(part 1 of 3)
# Autodesk Inventor assembly: Ensamblaje2
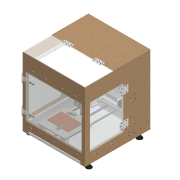
[picture p0: Inventor's stored thumbnail of the model, 180x180]
Saved by Autodesk Inventor 2020 (Build 240168000, 168)
## iProperties
Created: 2020-05-25
Part Number: Ensamblaje2
Document SubType Name: Assembly
Designer: Pipi
Author: Pipi
## Documents named in this file (110)
- C:\Users\Usuario\Desktop\Ensamble Ajuste Fino\Ensamblaje2.iam
- C:\Users\Usuario\Desktop\Ensamble Ajuste Fino\Culata.ipt
- C:\Users\Usuario\Desktop\Ensamble Ajuste Fino\Frente.ipt
- C:\Users\Usuario\Desktop\Ensamble Ajuste Fino\Lateral.ipt
- C:\Users\Usuario\Desktop\Ensamble Ajuste Fino\Soporte para Patas Regulables.ipt
- C:\Users\Usuario\Desktop\Ensamble Ajuste Fino\Pata regulable M6.ipt
- C:\Users\Usuario\Desktop\Ensamble Ajuste Fino\Guias de mesa.ipt
- C:\Users\Usuario\Desktop\Ensamble Ajuste Fino\Tornillo de mesa.ipt
- C:\Users\Usuario\Desktop\Ensamble Ajuste Fino\Buje para Tornillo.ipt
- C:\Users\Usuario\Desktop\Ensamble Ajuste Fino\Mesa.ipt
- C:\Users\Usuario\Desktop\Ensamble Ajuste Fino\Soporte de Buje.ipt
- C:\Users\Usuario\Desktop\Ensamble Ajuste Fino\Soporte de tuerca de mesa.ipt
- C:\Users\Usuario\Desktop\Ensamble Ajuste Fino\Buje para Guía.ipt
- C:\Users\Usuario\Desktop\Ensamble Ajuste Fino\Columna Derecha.ipt
- C:\Users\Usuario\Desktop\Ensamble Ajuste Fino\Columna Izquierda.ipt
- C:\Users\Usuario\Desktop\Ensamble Ajuste Fino\Guías de Vínculo Cabezal.ipt
- C:\Users\Usuario\Desktop\Ensamble Ajuste Fino\Tornillo de Vínculo Cabezal.ipt
- C:\Users\Usuario\Desktop\Ensamble Ajuste Fino\Travesaño Estructural.ipt
- C:\Users\Usuario\Desktop\Ensamble Ajuste Fino\Vertical Vìnculo Cabezal.ipt
- C:\Users\Usuario\Desktop\Ensamble Ajuste Fino\Bloque - Vinculo Cabezal.ipt
- C:\Users\Usuario\Desktop\Ensamble Ajuste Fino\Techo, Vínculo Cabezal.ipt
- C:\Users\Usuario\Desktop\Ensamble Ajuste Fino\Piso, Vínculo Cabezal.ipt
- C:\Users\Usuario\Desktop\Ensamble Ajuste Fino\Separador de Bujes.ipt
- C:\Users\Usuario\Desktop\Ensamble Ajuste Fino\Tapa para Buje.ipt
- C:\Users\Usuario\Desktop\Ensamble Ajuste Fino\motor DC.ipt
- C:\Users\Usuario\Desktop\Ensamble Ajuste Fino\Soporte de Motor.ipt
- C:\Users\Usuario\Desktop\Ensamble Ajuste Fino\Acople de soporte de motor.ipt
- C:\Users\Usuario\Desktop\Ensamble Ajuste Fino\Guías de Soporte de Motor.ipt
- C:\Users\Usuario\Desktop\Ensamble Ajuste Fino\Tornillo de Soporte de Motor.ipt
- C:\Users\Usuario\Desktop\Ensamble Ajuste Fino\Buje de Soporte de Motor.ipt
- C:\Users\Usuario\Desktop\Ensamble Ajuste Fino\Tornillo allen cabeza cilindrica M6x20mm.ipt
- C:\Users\Usuario\Desktop\Ensamble Ajuste Fino\Arandela Grower m6.ipt
- C:\Users\Usuario\Desktop\Ensamble Ajuste Fino\Tornillo Allen cabeza cilindrica M4x30mm.ipt
- C:\Users\Usuario\Desktop\Ensamble Ajuste Fino\Tornillo Allen cabeza cilindrica M4x16mm.ipt
- C:\Users\Usuario\Desktop\Ensamble Ajuste Fino\Nema 17.iam
- C:\Users\Usuario\Desktop\Ensamble Ajuste Fino\Acople de Motor PAP.ipt
- C:\Users\Usuario\Desktop\Ensamble Ajuste Fino\Tornillo Allen cabeza fresada M4x16mm.ipt
- C:\Users\Usuario\Desktop\Ensamble Ajuste Fino\Espaciador Sub Inferior.ipt
- C:\Users\Usuario\Desktop\Ensamble Ajuste Fino\Techo Espaciador Sub. Inferior.ipt
- C:\Users\Usuario\Desktop\Ensamble Ajuste Fino\Tornillo Allen cabeza botón M6x20mm.ipt
- C:\Users\Usuario\Desktop\Ensamble Ajuste Fino\Tornillo Allen cabeeza botón M3x8mm.ipt
- C:\Users\Usuario\Desktop\Ensamble Ajuste Fino\Espaciador Derecho.ipt
- C:\Users\Usuario\Desktop\Ensamble Ajuste Fino\Espaciador Izquierdo.ipt
- C:\Users\Usuario\Desktop\Ensamble Ajuste Fino\Techo Espaciador.ipt
- C:\Users\Usuario\Desktop\Ensamble Ajuste Fino\Tornillo Allen cabeza cilindrica M4x45mm.ipt
- C:\Users\Usuario\Desktop\Ensamble Ajuste Fino\Tornillo Allen cabeza cilindrica M4x20mm.ipt
- C:\Users\Usuario\Desktop\Ensamble Ajuste Fino\Tornillo Allen cabeza botón M4x20mm.ipt
- C:\Users\Usuario\Desktop\Ensamble Ajuste Fino\Final de Carrera.ipt
- C:\Users\Usuario\Desktop\Ensamble Ajuste Fino\Soporte de Final de Carrera - Eje X.ipt
- C:\Users\Usuario\Desktop\Ensamble Ajuste Fino\Tornillo Gusano Allen M3x16mm.ipt
- C:\Users\Usuario\Desktop\Ensamble Ajuste Fino\Herramienta Punta de Lanza.ipt
- C:\Users\Usuario\Desktop\Ensamble Ajuste Fino\Tornillo Allen cabeza botón M4x10mm.ipt
- C:\Users\Usuario\Desktop\Ensamble Ajuste Fino\Tuerca de mesa.ipt
- C:\Users\Usuario\Desktop\Ensamble Ajuste Fino\Arandela Plana Tipo A DIN 125 - M4.ipt
- C:\Users\Usuario\Desktop\Ensamble Ajuste Fino\Chaponete.ipt
- C:\Users\Usuario\Desktop\Ensamble Ajuste Fino\placa pcb 100x150mm.ipt
- C:\Users\Usuario\Desktop\Ensamble Ajuste Fino\Tornillo Allen cabeza fresada M3x20mm.ipt
- C:\Users\Usuario\Desktop\Ensamble Ajuste Fino\Arandela plana tipo A DIN 125 M6.ipt
- C:\Users\Usuario\Desktop\Ensamble Ajuste Fino\Tornillo Allen cabeza botón M6x16mm.ipt
- C:\Users\Usuario\Desktop\Ensamble Ajuste Fino\Tornillo allen cabeza boton M8x16mm.ipt
- C:\Users\Usuario\Desktop\Ensamble Ajuste Fino\Arandela Grower M8.ipt
- C:\Users\Usuario\Desktop\Ensamble Ajuste Fino\Soporte de Final de Carrera - Eje Y.ipt
- C:\Users\Usuario\Desktop\Ensamble Ajuste Fino\Placa de Mecanizado.ipt
- C:\Users\Usuario\Desktop\Ensamble Ajuste Fino\Esquina de bandeja.ipt
- C:\Users\Usuario\Desktop\Ensamble Ajuste Fino\Tornillo Allen cabeza cilindrica M4x35mm.ipt
- C:\Users\Usuario\Desktop\Ensamble Ajuste Fino\Tornillo Allen cabeza cilindrica M2x16mm.ipt
- C:\Users\Usuario\Desktop\Ensamble Ajuste Fino\Tapa de Mandril.ipt
- C:\Users\Usuario\Desktop\Ensamble Ajuste Fino\Remache POP Abierto con Rotura de Vástago D4.ipt
- C:\Users\Usuario\Desktop\Ensamble Ajuste Fino\Tornillo Allen gusano M6 para Motor.ipt
- C:\Users\Usuario\Desktop\Ensamble Ajuste Fino\Guía de Bandeja Der..ipt
- C:\Users\Usuario\Desktop\Ensamble Ajuste Fino\Guía de Bandeja Izq..ipt
- C:\Users\Usuario\Desktop\Ensamble Ajuste Fino\Bandeja.ipt
- C:\Users\Usuario\Desktop\Ensamble Ajuste Fino\Opción B - Sujeción Motor Paso a Paso\NEMA 17 90°.ipt
- C:\Users\Usuario\Desktop\Ensamble Ajuste Fino\Opción B - Sujeción Motor Paso a Paso\Estante para Soporte de Motor PaP.ipt
- C:\Users\Usuario\Desktop\Ensamble Ajuste Fino\Frente Carcasa.ipt
- C:\Users\Usuario\Desktop\Ensamble Ajuste Fino\Lateral Derecho Carcasa.ipt
- C:\Users\Usuario\Desktop\Ensamble Ajuste Fino\Lateral Izquierdo Carcasa.ipt
- C:\Users\Usuario\Desktop\Ensamble Ajuste Fino\Techo Carcasa.ipt
- C:\Users\Usuario\Desktop\Ensamble Ajuste Fino\Culata Carcaza.ipt
- C:\Users\Usuario\Desktop\Ensamble Ajuste Fino\Chapon.ipt
- C:\Users\Usuario\Desktop\Ensamble Ajuste Fino\Separador Lateral.ipt
- C:\Users\Usuario\Desktop\Ensamble Ajuste Fino\Cielo raso.ipt
- C:\Users\Usuario\Desktop\Ensamble Ajuste Fino\Puerta Lateral Izquierda.ipt
- C:\Users\Usuario\Desktop\Ensamble Ajuste Fino\Ala 1 Bisagra tipo Libro Grande.ipt
- C:\Users\Usuario\Desktop\Ensamble Ajuste Fino\Ala 2 Bisagra tipo Libro Grande.ipt
- C:\Users\Usuario\Desktop\Ensamble Ajuste Fino\Ala 1 Bisagra tipo T.ipt
- C:\Users\Usuario\Desktop\Ensamble Ajuste Fino\Ala 2 Bisagra tipo T.ipt
- C:\Users\Usuario\Desktop\Ensamble Ajuste Fino\Distanciador para Laterales.ipt
- C:\Users\Usuario\Desktop\Ensamble Ajuste Fino\Ala 1 Bisagra tipo Libro Chica.ipt
- C:\Users\Usuario\Desktop\Ensamble Ajuste Fino\Ala 2 Bisagra tipo Libro Chica.ipt
- C:\Users\Usuario\Desktop\Ensamble Ajuste Fino\Soporte L.ipt
- C:\Users\Usuario\Desktop\Ensamble Ajuste Fino\Tuerca remache m4.ipt
- C:\Users\Usuario\Desktop\Ensamble Ajuste Fino\Chapa Base.ipt
- C:\Users\Usuario\Documents\Inventor\Content Center Files\R2020\en-US\ISO 4032(2)\ISO 4032 - M6 - ISO.ipt
- C:\Users\Usuario\Documents\Inventor\Content Center Files\R2020\en-US\ISO 4032(2)\ISO 4032 - M4 - ISO.ipt
- C:\Users\Usuario\Desktop\Ensamble Ajuste Fino\Tornillo allen cabeza boton M5x10mm.ipt
- C:\Users\Usuario\Desktop\Ensamble Ajuste Fino\Arandela plana tipo A DIN 125-M5.ipt
- C:\Users\Usuario\Documents\Inventor\Content Center Files\R2020\en-US\ISO 4032(2)\ISO 4032 - M5 - ISO.ipt
- C:\Users\Usuario\Desktop\Ensamble Ajuste Fino\Tornillo allen cabeza boton M5x16mm.ipt
- C:\Users\Usuario\Desktop\Ensamble Ajuste Fino\Puerta Frontal.ipt
- C:\Users\Usuario\Desktop\Ensamble Ajuste Fino\Puerta Lateral Derecha.ipt
- C:\Users\Usuario\Desktop\Ensamble Ajuste Fino\Puerta de Inspección.ipt
- C:\Users\Usuario\Desktop\Ensamble Ajuste Fino\Soporte para culata carcasa.ipt
- C:\Users\Usuario\Desktop\Ensamble Ajuste Fino\Tornillo Allen cabeza botón M4x16mm.ipt
- C:\Users\Usuario\Documents\Inventor\Content Center Files\R2020\en-US\ISO 4032(2)\ISO 4032 - M2 - ISO.ipt
- C:\Users\Usuario\Documents\Inventor\Content Center Files\R2020\en-US\ISO 4032(2)\ISO 4032 - M3 - ISO.ipt
- C:\Users\Usuario\Desktop\Ensamble Ajuste Fino\Kit de sujecion 2.ipt
- C:\Users\Usuario\Desktop\Ensamble Ajuste Fino\Kit sugecion 1.ipt
- C:\Users\Usuario\Desktop\Ensamble Ajuste Fino\Eslabon cadena portacable.ipt
- C:\Users\Usuario\Desktop\Ensamble Ajuste Fino\Tornillo Allen cabeeza botón M3x16mm.ipt
## Components (623 placed, 109 different names)
1. Culata:1 — Coincidencia:4, Coincidencia:91, Coincidencia:92, Coincidencia:93, Coincidencia:94, Coincidencia:95, Coincidencia:96, Coincidencia:148, Nivelación:20, Coincidencia:186, Coincidencia:220, Mate:275, Nivelación:38, Coincidencia:292, Insertar:469, Insertar:470
2. Frente:1 — Coincidencia:21, Coincidencia:22, Nivelación:12, Nivelación:16, Nivelación:17, Coincidencia:154, Insertar:236, Insertar:285, Coincidencia:193, Insertar:286, Coincidencia:274, Coincidencia:400
3. Lateral:1 — Coincidencia:4, Insertar:35, Insertar:36, Insertar:37, Insertar:38, Insertar:71, Insertar:72, Coincidencia:89, Coincidencia:90, Nivelación:12, Insertar:236, Nivelación:39, Mate:301, Mate:302, Mate:303, Coincidencia:385, Nivelación:58, Insertar:487, Insertar:488, Insertar:489
4. Lateral:2 — Nivelación:16, Nivelación:17, Coincidencia:154, Insertar:234, Insertar:235, Insertar:237, Insertar:238, Insertar:239, Coincidencia:155, Insertar:254, Coincidencia:170, Insertar:308, Mate:304, Mate:305, Mate:306, Coincidencia:383, Nivelación:57, Insertar:490, Insertar:491, Insertar:492
5. Soporte para Patas Regulables:1 — Insertar:2, Insertar:72, Coincidencia:90, Insertar:77, Insertar:78
6. Soporte para Patas Regulables:2 — Insertar:3, Insertar:73, Insertar:74, Insertar:239
7. Soporte para Patas Regulables:3 — Insertar:4, Insertar:75, Insertar:76, Insertar:254, Coincidencia:170
8. Soporte para Patas Regulables:4 — Insertar:1, Insertar:71, Coincidencia:89, Insertar:79, Insertar:80
9. Pata regulable M6:1 — Insertar:1
10. Pata regulable M6:2 — Insertar:2
11. Pata regulable M6:3 — Insertar:3
12. Pata regulable M6:4 — Insertar:4
13. Guias de mesa:1 — Insertar:285, Coincidencia:190, Coincidencia:212, Insertar:324, Insertar:330
14. Guias de mesa:2 — Coincidencia:193, Insertar:286, Coincidencia:194, Insertar:323, Insertar:329
15. Tornillo de mesa:1 — Insertar:278, Coincidencia:216
16. Buje para Tornillo:1 — Coincidencia:21, Coincidencia:22, Insertar:278
17. Mesa:1 — Coincidencia:197, Coincidencia:198, Coincidencia:200, Coincidencia:203, Coincidencia:205, Coincidencia:206, Coincidencia:208, Coincidencia:209, Coincidencia:210, Coincidencia:217, Coincidencia:218, Coincidencia:274, Mate:275, Nivelación:36, Coincidencia:280, Nivelación:37, Mate:363, Mate:364, Mate:368, Mate:369, Mate:370, Mate:371
18. Soporte de Buje:1 — Coincidencia:211, Nivelación:22, Coincidencia:218, Insertar:299, Insertar:300, Insertar:301, Insertar:302, Coincidencia:251, Coincidencia:256
19. Soporte de Buje:2 — Coincidencia:213, Nivelación:21, Coincidencia:217, Insertar:291, Insertar:292, Insertar:293, Insertar:294, Coincidencia:252, Coincidencia:254
20. Soporte de Buje:3 — Coincidencia:198, Coincidencia:203, Coincidencia:206, Coincidencia:215, Nivelación:24, Insertar:287, Insertar:288, Insertar:289, Insertar:290, Coincidencia:253, Coincidencia:255
21. Soporte de Buje:4 — Coincidencia:197, Coincidencia:200, Coincidencia:205, Coincidencia:214, Nivelación:23, Insertar:295, Insertar:296, Insertar:297, Insertar:298, Coincidencia:250, Coincidencia:257
22. Soporte de tuerca de mesa:1 — Coincidencia:208, Coincidencia:209, Coincidencia:210, Coincidencia:216, Insertar:303, Insertar:304, Insertar:305, Insertar:306, Insertar:307, Coincidencia:219, Coincidencia:423, Nivelación:60
23. Buje para Guía:1 — Coincidencia:212, Coincidencia:213, Nivelación:21, Insertar:341, Insertar:344
24. Buje para Guía:2 — Coincidencia:190, Coincidencia:211, Nivelación:22, Insertar:346, Insertar:349
25. Buje para Guía:3 — Coincidencia:215, Nivelación:24, Insertar:342, Insertar:343
26. Buje para Guía:4 — Coincidencia:194, Coincidencia:214, Nivelación:23, Insertar:340, Insertar:345
27. Columna Derecha:1 — Coincidencia:40, Coincidencia:41, Coincidencia:44, Nivelación:7, Coincidencia:46, Nivelación:8, Insertar:128, Insertar:129, Insertar:170, Insertar:172, Insertar:173, Coincidencia:116, Insertar:174, Insertar:175, Insertar:205, Insertar:206, Insertar:207, Insertar:208, Insertar:237, Insertar:238, Insert:442, Mate:348, Flush:42, Coincidencia:384
28. Columna Izquierda:1 — Coincidencia:37, Coincidencia:42, Coincidencia:43, Coincidencia:45, Coincidencia:47, Coincidencia:48, Insertar:126, Insertar:127, Coincidencia:126, Coincidencia:127, Coincidencia:128, Insertar:201, Insertar:202, Insertar:203, Insertar:204, Coincidencia:386
29. Guías de Vínculo Cabezal:1 — Coincidencia:46, Nivelación:8, Coincidencia:64, Coincidencia:65, Coincidencia:66, Coincidencia:73, Coincidencia:74, Insertar:334, Insertar:338
30. Guías de Vínculo Cabezal:2 — Coincidencia:45, Nivelación:7, Coincidencia:61, Coincidencia:62, Coincidencia:63, Coincidencia:71, Coincidencia:72, Insertar:332, Insertar:336
31. Tornillo de Vínculo Cabezal:1 — Insertar:17, Coincidencia:117, Insertar:176, Coincidencia:173
32. Travesaño Estructural:1 — Coincidencia:37, Coincidencia:40, Coincidencia:41, Coincidencia:42, Coincidencia:43, Coincidencia:44, Insertar:747, Insertar:748, Insertar:749, Insertar:750
33. Buje para Tornillo:2 — Coincidencia:47, Coincidencia:48, Insertar:17
34. Vertical Vìnculo Cabezal:1 — Coincidencia:53, Coincidencia:54, Coincidencia:55, Coincidencia:56, Insertar:138, Insertar:139, Insertar:140, Insertar:141, Insertar:142, Insertar:143, Insertar:144, Insertar:145, Coincidencia:118, Coincidencia:120
35. Bloque - Vinculo Cabezal:1 — Coincidencia:118, Coincidencia:119, Coincidencia:120, Insertar:177, Insertar:178, Insertar:179, Insertar:180, Insertar:181, Insertar:182, Coincidencia:125, Coincidencia:139, Coincidencia:171, Coincidencia:172, Insertar:255, Coincidencia:174, Insertar:852, Insertar:853
36. Techo, Vínculo Cabezal:1 — Coincidencia:55, Coincidencia:56, Coincidencia:105, Coincidencia:106, Coincidencia:107, Coincidencia:108, Coincidencia:109, Coincidencia:110, Coincidencia:119, Insertar:279, Insertar:280, Insertar:364, Insertar:365, Insertar:366, Insertar:367, Coincidencia:271, Insertar:411, Coincidencia:291
37. Piso, Vínculo Cabezal:1 — Coincidencia:53, Coincidencia:54, Coincidencia:79, Coincidencia:80, Insertar:368, Insertar:369, Insertar:370, Insertar:371, Coincidencia:272
38. Buje para Guía:5 — Coincidencia:64, Coincidencia:70, Insertar:178
39. Buje para Guía:6 — Coincidencia:66, Coincidencia:69
40. Buje para Guía:7 — Coincidencia:62, Coincidencia:68, Insertar:177
41. Buje para Guía:8 — Coincidencia:61, Coincidencia:67
42. Separador de Bujes:1 — Coincidencia:65, Coincidencia:69, Coincidencia:70
43. Separador de Bujes:2 — Coincidencia:63, Coincidencia:67, Coincidencia:68
44. Tapa para Buje:1 — Coincidencia:72, Insertar:148, Insertar:149, Insertar:181
45. Tapa para Buje:2 — Coincidencia:74, Insertar:154, Insertar:155, Insertar:180
46. Tapa para Buje:3 — Coincidencia:73, Insertar:150, Insertar:151, Insertar:182
47. Tapa para Buje:4 — Coincidencia:71, Insertar:152, Insertar:153, Insertar:179
48. motor DC:1 — Coincidencia:270, Nivelación:31, Coincidencia:273, Nivelación:32, Mate:294, Mate:295
49. Acople de soporte de motor:1 — Coincidencia:263, Coincidencia:264, Insertar:389, Coincidencia:265, Insertar:390, Coincidencia:266, Insertar:391, Coincidencia:267, Insertar:392, Coincidencia:268, Insertar:393, Insertar:394, Insertar:395, Insertar:396, Insertar:397
50. Guías de Soporte de Motor:1 — Coincidencia:180, Insertar:280, Insertar:381, Insertar:383, Coincidencia:259, Coincidencia:263
51. Guías de Soporte de Motor:2 — Coincidencia:182, Insertar:279, Insertar:380, Insertar:382, Coincidencia:258, Coincidencia:264
52. Buje para Tornillo:3 — Coincidencia:79, Coincidencia:80, Insertar:24
53. Tornillo de Soporte de Motor:1 — Insertar:24, Coincidencia:290, Insertar:410
54. Buje de Soporte de Motor:1 — Insertar:266, Coincidencia:258, Insertar:391, Coincidencia:272
55. Buje de Soporte de Motor:2 — Coincidencia:180, Insertar:268, Insertar:390
56. Tornillo allen cabeza cilindrica M6x20mm:5 — Insertar:235
57. Tornillo allen cabeza cilindrica M6x20mm:6
58. Tornillo allen cabeza cilindrica M6x20mm:7 — Insertar:308, Coincidencia:220
59. Tornillo allen cabeza cilindrica M6x20mm:10 — Insertar:38
60. Tornillo allen cabeza cilindrica M6x20mm:15 — Insertar:37, Coincidencia:148
61. Tornillo allen cabeza cilindrica M6x20mm:16 — Insertar:35
62. Tornillo allen cabeza cilindrica M6x20mm:17 — Insertar:36
63. Tornillo allen cabeza cilindrica M6x20mm:20 — Insertar:234
64. Arandela Grower m6:1 — Insertar:320, Insert:429
65. Arandela Grower m6:2 — Insertar:322, Insert:428
66. Arandela Grower m6:3 — Insertar:326, Insert:427
67. Arandela Grower m6:4 — Insertar:328, Insert:426
68. Tornillo Allen cabeza cilindrica M4x30mm:1 — Insertar:290
69. Tornillo Allen cabeza cilindrica M4x30mm:2 — Insertar:291
70. Tornillo Allen cabeza cilindrica M4x30mm:3 — Insertar:299
71. Tornillo Allen cabeza cilindrica M4x30mm:4 — Insertar:301
72. Tornillo Allen cabeza cilindrica M4x30mm:5 — Insertar:298
73. Tornillo Allen cabeza cilindrica M4x30mm:6 — Insertar:287
74. Tornillo Allen cabeza cilindrica M4x30mm:7 — Insertar:294
75. Tornillo Allen cabeza cilindrica M4x30mm:8 — Insertar:302
76. Tornillo Allen cabeza cilindrica M4x30mm:9 — Insertar:288
77. Tornillo Allen cabeza cilindrica M4x30mm:10 — Insertar:300
78. Tornillo Allen cabeza cilindrica M4x30mm:15 — Insertar:293
79. Tornillo Allen cabeza cilindrica M4x30mm:16 — Insertar:292
80. Tornillo Allen cabeza cilindrica M4x30mm:17 — Insertar:296
81. Tornillo Allen cabeza cilindrica M4x30mm:18 — Insertar:289
82. Tornillo Allen cabeza cilindrica M4x30mm:19 — Insertar:297
83. Tornillo Allen cabeza cilindrica M4x30mm:20 — Insertar:295
84. Tornillo Allen cabeza cilindrica M4x16mm:1 — Insertar:83, Coincidencia:99
85. Tornillo Allen cabeza cilindrica M4x16mm:2 — Insertar:86
86. Tornillo Allen cabeza cilindrica M4x16mm:3 — Insertar:84
87. Tornillo Allen cabeza cilindrica M4x16mm:4 — Insertar:306
88. Tornillo Allen cabeza cilindrica M4x16mm:5 — Insertar:303
89. Tornillo Allen cabeza cilindrica M4x16mm:6 — Insertar:85
90. Nema 17:1 [sub-assembly] — Insertar:82, Coincidencia:99
91. Nema 17:2 [sub-assembly] — Coincidencia:116, Insertar:174, Insertar:175, Coincidencia:117, Mate:345, Mate:346, Mate:347
92. Nema 17:3 [sub-assembly] — Coincidencia:115, Insertar:169, Coincidencia:290
93. Acople de Motor PAP:2 — Insertar:176, Coincidencia:125
94. Acople de Motor PAP:1 — Nivelación:20, Coincidencia:186
95. Acople de Motor PAP:3 — Coincidencia:115, Insertar:410
96. Tornillo Allen cabeza fresada M4x16mm:1 — Insertar:77
97. Tornillo Allen cabeza fresada M4x16mm:2 — Insertar:78
98. Tornillo Allen cabeza fresada M4x16mm:3 — Insertar:79
99. Tornillo Allen cabeza fresada M4x16mm:4 — Insertar:74, Coincidencia:155
100. Tornillo Allen cabeza fresada M4x16mm:5 — Insertar:80
101. Tornillo Allen cabeza fresada M4x16mm:6 — Insertar:76
102. Tornillo Allen cabeza fresada M4x16mm:7 — Insertar:75
103. Tornillo Allen cabeza fresada M4x16mm:8 — Insertar:73
104. Espaciador Sub Inferior:1 — Coincidencia:92, Coincidencia:93, Coincidencia:94, Coincidencia:97, Insertar:91
105. Espaciador Sub Inferior:2 — Coincidencia:91, Coincidencia:95, Coincidencia:96, Mate:293
106. Techo Espaciador Sub. Inferior:1 — Insertar:82, Insertar:83, Insertar:84, Insertar:85, Insertar:86, Coincidencia:97, Insertar:91, Insert:412, Insert:413, Insert:414, Insert:415
107. Tornillo Allen cabeza cilindrica M4x16mm:7 — Insertar:305
108. Tornillo Allen cabeza cilindrica M4x16mm:8 — Insertar:304
109. Arandela Grower m6:5 — Insertar:372, Insertar:373
110. Arandela Grower m6:6 — Insertar:374, Insertar:375
111. Arandela Grower m6:7 — Insertar:109, Insertar:331
112. Arandela Grower m6:8 — Insertar:124, Insertar:128
113. Arandela Grower m6:9 — Insertar:103, Insertar:337
114. Arandela Grower m6:10 — Insertar:107, Insertar:333
115. Arandela Grower m6:11 — Insertar:122, Insertar:127
116. Arandela Grower m6:12 — Insertar:125, Insertar:129
117. Arandela Grower m6:13 — Insertar:100, Insertar:335
118. Arandela Grower m6:14 — Insertar:123, Insertar:126
119. Arandela Grower m6:15 — Insertar:378, Insertar:379
120. Arandela Grower m6:16 — Insertar:376, Insertar:377
121. Tornillo Allen cabeza botón M6x20mm:3 — Insertar:100
122. Tornillo Allen cabeza botón M6x20mm:4 — Insertar:107
123. Tornillo Allen cabeza botón M6x20mm:5 — Insertar:374
124. Tornillo Allen cabeza botón M6x20mm:6 — Insertar:109
125. Tornillo Allen cabeza botón M6x20mm:7 — Insertar:372
126. Tornillo Allen cabeza botón M6x20mm:8 — Insertar:103
127. Tornillo Allen cabeza botón M6x20mm:9 — Insertar:376
128. Tornillo Allen cabeza botón M6x20mm:10 — Insertar:378
129. Tornillo Allen cabeza botón M6x20mm:11 — Insertar:122
130. Tornillo Allen cabeza botón M6x20mm:12 — Insertar:124
131. Tornillo Allen cabeza botón M6x20mm:18 — Insertar:138
132. Tornillo Allen cabeza botón M6x20mm:20 — Insertar:125
133. Tornillo Allen cabeza botón M6x20mm:21 — Insertar:123
134. Tornillo Allen cabeza botón M6x20mm:22 — Insertar:144
135. Tornillo Allen cabeza botón M6x20mm:23 — Insertar:143
136. Tornillo Allen cabeza botón M6x20mm:24 — Insertar:140
137. Tornillo Allen cabeza botón M6x20mm:25 — Insertar:139
138. Tornillo Allen cabeza botón M6x20mm:26 — Insertar:145
139. Tornillo Allen cabeza botón M6x20mm:27 — Insertar:142
140. Tornillo Allen cabeza botón M6x20mm:28 — Insertar:141
141. Tornillo Allen cabeeza botón M3x8mm:1 — Insertar:153
142. Tornillo Allen cabeeza botón M3x8mm:2 — Insertar:150
143. Tornillo Allen cabeeza botón M3x8mm:3 — Insertar:152
144. Tornillo Allen cabeeza botón M3x8mm:4 — Insertar:154
145. Tornillo Allen cabeeza botón M3x8mm:5 — Insertar:155
146. Tornillo Allen cabeeza botón M3x8mm:6 — Insertar:151
147. Tornillo Allen cabeeza botón M3x8mm:7 — Insertar:148
148. Tornillo Allen cabeeza botón M3x8mm:8 — Insertar:149
149. Espaciador Derecho:1 — Coincidencia:108, Coincidencia:109, Coincidencia:110, Coincidencia:112, Coincidencia:113
150. Espaciador Izquierdo:1 — Coincidencia:105, Coincidencia:106, Coincidencia:107, Coincidencia:111, Coincidencia:114
151. Techo Espaciador:1 — Coincidencia:111, Coincidencia:112, Coincidencia:113, Coincidencia:114, Insertar:165, Insertar:166, Insertar:167, Insertar:168, Insertar:169, Insertar:185, Insertar:186, Insertar:187, Insertar:217, Insertar:218, Insertar:219, Insertar:220
152. Tornillo Allen cabeza cilindrica M4x45mm:1 — Insertar:186
153. Tornillo Allen cabeza cilindrica M4x45mm:3 — Insertar:185
154. Tornillo Allen cabeza cilindrica M4x45mm:4 — Insertar:187
155. Tornillo Allen cabeza cilindrica M4x20mm:1 — Insertar:167
156. Tornillo Allen cabeza cilindrica M4x20mm:2 — Insertar:166
157. Tornillo Allen cabeza cilindrica M4x20mm:3 — Insertar:165
158. Tornillo Allen cabeza cilindrica M4x20mm:4 — Insertar:168
159. Tornillo Allen cabeza botón M4x20mm:3 — Insertar:173
160. Tornillo Allen cabeza botón M4x20mm:4 — Insertar:172
161. Tornillo Allen cabeza botón M4x20mm:5 — Insertar:170
162. Final de Carrera:1 — Insertar:398, Coincidencia:277, Insert:420, Insert:421
163. Final de Carrera:2 — Coincidencia:129, Coincidencia:130, Coincidencia:131, Coincidencia:139, Insert:418, Insert:419
164. Final de Carrera:3 — Insertar:411, Coincidencia:291, Insert:416, Insert:417
165. Soporte de Final de Carrera - Eje X:1 — Coincidencia:126, Coincidencia:127, Coincidencia:128, Coincidencia:129, Coincidencia:130, Coincidencia:131, Insertar:213, Insertar:214, Coincidencia:420, Coincidencia:422
166. Arandela Grower m6:17 — Insertar:206, Insert:432
167. Arandela Grower m6:18 — Insertar:208, Insert:433
168. Arandela Grower m6:19 — Insertar:203, Insert:424
169. Arandela Grower m6:20 — Insertar:202, Insert:425
170. Arandela Grower m6:21 — Insertar:201, Insert:422
171. Arandela Grower m6:22 — Insertar:207, Insert:430
172. Arandela Grower m6:23 — Insertar:205, Insert:431
173. Arandela Grower m6:24 — Insertar:204, Insert:423
174. Tornillo Gusano Allen M3x16mm:1 — Coincidencia:171, Nivelación:18
175. Tornillo Gusano Allen M3x16mm:2 — Coincidencia:172, Nivelación:19
176. Tornillo Gusano Allen M3x16mm:3 — Flush:41, Mate:344
177. Tornillo Gusano Allen M3x16mm:4 — Insertar:257, Coincidencia:219
178. Tornillo Allen cabeeza botón M3x8mm:9 — Insertar:214
179. Tornillo Allen cabeeza botón M3x8mm:10 — Insertar:213
180. Tornillo Allen cabeza cilindrica M4x45mm:1 — Insertar:218
181. Tornillo Allen cabeza cilindrica M4x45mm:2 — Insertar:219
182. Tornillo Allen cabeza cilindrica M4x45mm:3 — Insertar:220
183. Tornillo Allen cabeza cilindrica M4x45mm:4 — Insertar:217
184. Tornillo Allen cabeeza botón M3x8mm:11 — Insertar:266, Coincidencia:267
185. Tornillo Allen cabeeza botón M3x8mm:12 — Insertar:270, Coincidencia:268
186. Herramienta Punta de Lanza:1 — Coincidencia:273, Nivelación:32
187. Tuerca de mesa:2 — Insertar:257, Insertar:307, Flush:41, Mate:344
188. Tuerca de mesa:3 — Coincidencia:173, Insertar:255, Coincidencia:174, Nivelación:18, Nivelación:19
189. Buje de Soporte de Motor:5 — Coincidencia:182, Insertar:271, Insertar:389, Coincidencia:271
190. Buje de Soporte de Motor:6 — Insertar:270, Coincidencia:259, Insertar:392
191. Tornillo Allen cabeeza botón M3x8mm:13 — Insertar:268, Coincidencia:266
192. Tornillo Allen cabeeza botón M3x8mm:16 — Insertar:271, Coincidencia:265
193. Arandela plana tipo A DIN 125 M6:1 — Insertar:331, Insertar:332
194. Arandela plana tipo A DIN 125 M6:2 — Insertar:328, Insertar:329
195. Arandela plana tipo A DIN 125 M6:3 — Insertar:326, Insertar:330
196. Arandela plana tipo A DIN 125 M6:4 — Insertar:333, Insertar:334
197. Arandela plana tipo A DIN 125 M6:5 — Insertar:335, Insertar:336
198. Arandela plana tipo A DIN 125 M6:6 — Insertar:337, Insertar:338
199. Arandela plana tipo A DIN 125 M6:7 — Insertar:322, Insertar:323
200. Arandela plana tipo A DIN 125 M6:8 — Insertar:320, Insertar:324
201. Tapa para Buje:5 — Insertar:349, Coincidencia:251, Insertar:350, Insertar:351
202. Tapa para Buje:6 — Insertar:342, Coincidencia:253, Insertar:353, Insertar:355
203. Tapa para Buje:7 — Insertar:340, Coincidencia:250, Insertar:347, Insertar:348
204. Tapa para Buje:8 — Insertar:343, Coincidencia:255, Insertar:358, Insertar:359
205. Tapa para Buje:9 — Insertar:341, Coincidencia:252, Insertar:352, Insertar:354
206. Tapa para Buje:10 — Insertar:344, Coincidencia:254, Insertar:356, Insertar:357
207. Tapa para Buje:11 — Insertar:346, Coincidencia:256, Insertar:360, Insertar:363
208. Tapa para Buje:12 — Insertar:345, Coincidencia:257, Insertar:361, Insertar:362
209. Tornillo Allen cabeeza botón M3x8mm:17 — Insertar:347
210. Tornillo Allen cabeeza botón M3x8mm:18 — Insertar:363
211. Tornillo Allen cabeeza botón M3x8mm:19 — Insertar:362
212. Tornillo Allen cabeeza botón M3x8mm:20 — Insertar:356
213. Tornillo Allen cabeeza botón M3x8mm:21 — Insertar:355
214. Tornillo Allen cabeeza botón M3x8mm:22 — Insertar:354
215. Tornillo Allen cabeeza botón M3x8mm:23 — Insertar:361
216. Tornillo Allen cabeeza botón M3x8mm:24 — Insertar:360
217. Tornillo Allen cabeeza botón M3x8mm:25 — Insertar:348
218. Tornillo Allen cabeeza botón M3x8mm:26 — Insertar:359
219. Tornillo Allen cabeeza botón M3x8mm:27 — Insertar:358
220. Tornillo Allen cabeeza botón M3x8mm:28 — Insertar:357
221. Tornillo Allen cabeeza botón M3x8mm:29 — Insertar:353
222. Tornillo Allen cabeeza botón M3x8mm:30 — Insertar:352
223. Tornillo Allen cabeeza botón M3x8mm:31 — Insertar:351
224. Tornillo Allen cabeeza botón M3x8mm:32 — Insertar:350
225. Tornillo Allen cabeza botón M6x16mm:1 — Insertar:367
226. Tornillo Allen cabeza botón M6x16mm:2 — Insertar:366
227. Tornillo Allen cabeza botón M6x16mm:3 — Insertar:365
228. Tornillo Allen cabeza botón M6x16mm:4 — Insertar:364
229. Tornillo Allen cabeza botón M6x16mm:5 — Insertar:371
230. Tornillo Allen cabeza botón M6x16mm:6 — Insertar:370
231. Tornillo Allen cabeza botón M6x16mm:7 — Insertar:369
232. Tornillo Allen cabeza botón M6x16mm:8 — Insertar:368
233. Arandela plana tipo A DIN 125 M6:9 — Insertar:375, Insertar:380
234. Arandela plana tipo A DIN 125 M6:10 — Insertar:373, Insertar:381
235. Arandela plana tipo A DIN 125 M6:11 — Insertar:377, Insertar:382
236. Arandela plana tipo A DIN 125 M6:12 — Insertar:379, Insertar:383
237. Soporte de Motor:1 — Insertar:397, Coincidencia:269, Coincidencia:270, Nivelación:31, Flush:40, Mate:296
238. Tornillo allen cabeza boton M8x16mm:1 — Insertar:388
239. Tornillo allen cabeza boton M8x16mm:2 — Insertar:387, Coincidencia:269
240. Tornillo allen cabeza boton M8x16mm:3 — Insertar:386
241. Tornillo allen cabeza boton M8x16mm:4 — Insertar:385
242. Arandela Grower M8:1 — Insertar:386, Insertar:393
243. Arandela Grower M8:2 — Insertar:387, Insertar:394
244. Arandela Grower M8:3 — Insertar:388, Insertar:395
245. Arandela Grower M8:4 — Insertar:385, Insertar:396
246. Soporte de Final de Carrera - Eje Y:1 — Insertar:398, Coincidencia:277, Nivelación:38, Coincidencia:292, Nivelación:39, Insertar:846, Insertar:847, Coincidencia:412, Coincidencia:414
247. Placa de Mecanizado:1 — Coincidencia:279, Nivelación:34, Nivelación:35, Nivelación:36, Coincidencia:280, Nivelación:37
248. placa pcb 100x150mm:1 — Coincidencia:279, Nivelación:34, Nivelación:35
249. Esquina de bandeja:1 — Mate:307, Mate:308, Mate:309, Mate:311, Mate:340
250. Tornillo Allen cabeza cilindrica M4x35mm:1 — Insert:412
251. Tornillo Allen cabeza cilindrica M4x35mm:2 — Insert:415, Mate:293
252. Tornillo Allen cabeza cilindrica M4x35mm:3 — Insert:414
253. Tornillo Allen cabeza cilindrica M4x35mm:4 — Insert:413
254. Tornillo Allen cabeza cilindrica M2x16mm:1 — Insert:417
255. Tornillo Allen cabeza cilindrica M2x16mm:2 — Insert:416
256. Tornillo Allen cabeza cilindrica M2x16mm:3 — Insert:418, Coincidencia:419
257. Tornillo Allen cabeza cilindrica M2x16mm:4 — Insert:419, Coincidencia:421
258. Tornillo Allen cabeza cilindrica M2x16mm:6 — Insert:420, Coincidencia:413
259. Tornillo Allen cabeza cilindrica M2x16mm:7 — Insert:421, Coincidencia:411
260. Tapa de Mandril:1 — Mate:294, Mate:295
261. Tornillo Allen cabeza botón M6x20mm:29 — Insert:427
262. Tornillo Allen cabeza botón M6x20mm:30 — Insert:426
263. Tornillo Allen cabeza botón M6x20mm:31 — Insert:429
264. Tornillo Allen cabeza botón M6x20mm:32 — Insert:428
265. Tornillo Allen cabeza botón M6x20mm:33 — Insert:430
266. Tornillo Allen cabeza botón M6x20mm:34 — Insert:431
267. Tornillo Allen cabeza botón M6x20mm:35 — Insert:433
268. Tornillo Allen cabeza botón M6x20mm:36 — Insert:432
269. Tornillo Allen cabeza botón M6x20mm:37 — Insert:422
270. Tornillo Allen cabeza botón M6x20mm:38 — Insert:423
271. Tornillo Allen cabeza botón M6x20mm:39 — Insert:424
272. Tornillo Allen cabeza botón M6x20mm:40 — Insert:425
273. Remache POP Abierto con Rotura de Vástago D4:5 — Insert:459
274. Remache POP Abierto con Rotura de Vástago D4:6 — Insert:451
275. Remache POP Abierto con Rotura de Vástago D4:7 — Insert:456
276. Remache POP Abierto con Rotura de Vástago D4:8 — Insert:449, Mate:373
277. Tornillo Allen cabeza botón M4x20mm:6 — Insert:442
278. Tornillo Allen gusano M6 para Motor:1 — Flush:40, Mate:296
279. Guía de Bandeja Izq.:1 — Mate:301, Mate:302, Mate:303, Insert:443, Insert:444, Insert:445, Mate:372, Mate:373
280. Guía de Bandeja Der.:1 — Mate:304, Mate:305, Mate:306, Insert:446, Insert:447, Insert:448, Mate:374
281. Tornillo Allen cabeza botón M4x10mm:1 — Insert:448
282. Tornillo Allen cabeza botón M4x10mm:2 — Insert:447
283. Tornillo Allen cabeza botón M4x10mm:3 — Insert:446
284. Tornillo Allen cabeza botón M4x10mm:4 — Insert:443
285. Tornillo Allen cabeza botón M4x10mm:5 — Insert:445
286. Tornillo Allen cabeza botón M4x10mm:6 — Insert:444
287. Bandeja:1 — Mate:307, Mate:308, Mate:309, Mate:311, Mate:312, Mate:319, Mate:320, Mate:321, Insert:449, Insert:451, Mate:331, Mate:333, Insert:454, Insert:455, Mate:337, Mate:338, Mate:339, Mate:340, Insert:456, Insert:457, Insert:458, Insert:459, Mate:372
288. Esquina de bandeja:2 — Mate:312, Mate:319, Mate:320, Mate:321, Mate:337
289. Esquina de bandeja:3 — Mate:331, Mate:338, Mate:374
290. Esquina de bandeja:4 — Mate:333, Mate:339
291. Remache POP Abierto con Rotura de Vástago D4:9 — Insert:457
292. Remache POP Abierto con Rotura de Vástago D4:10 — Insert:454
293. Remache POP Abierto con Rotura de Vástago D4:11 — Insert:458
294. Remache POP Abierto con Rotura de Vástago D4:12 — Insert:455
295. NEMA 17 90°:1 — Mate:345, Mate:346, Mate:347, Mate:349
296. Estante para Soporte de Motor PaP:1 — Mate:348, Flush:42, Mate:349
297. Chaponete:3 — Mate:360, Flush:49, Insert:466, Flush:50, Mate:364
298. Tornillo Allen cabeza fresada M3x20mm:4 — Insert:466, Mate:371
299. Arandela Plana Tipo A DIN 125 - M4:3 — Insert:465, Mate:360
300. Tornillo Allen cabeza cilindrica M4x20mm:7 — Insert:465, Mate:361, Mate:362, Mate:363
301. Chaponete:5 — Mate:365, Flush:51, Flush:52, Insert:468, Mate:369
302. Tornillo Allen cabeza fresada M3x20mm:6 — Insert:468, Mate:370
303. Tornillo Allen cabeza cilindrica M4x20mm:9 — Insert:467, Mate:366, Mate:367, Mate:368
304. Arandela Plana Tipo A DIN 125 - M4:5 — Insert:467, Mate:365
305. Frente Carcasa:1 — Coincidencia:375, Coincidencia:376, Nivelación:53, Coincidencia:377, Coincidencia:378, Nivelación:54, Insertar:472, Coincidencia:400, Insertar:543, Insertar:544, Insertar:639, Insertar:640, Insertar:693, Insertar:694, Insertar:695, Insertar:696, Insertar:697, Insertar:698, Insertar:699, Ángulo:7
306. Lateral Derecho Carcasa:1 — Coincidencia:375, Coincidencia:376, Nivelación:53, Coincidencia:379, Nivelación:55, Nivelación:56, Coincidencia:380, Coincidencia:381, Insertar:471, Insertar:473, Insertar:474, Insertar:475, Insertar:476, Insertar:529, Insertar:530, Insertar:531, Insertar:532, Insertar:541, Insertar:542, Insertar:546, Nivelación:59, Insertar:568, Insertar:569, Insertar:570, Insertar:571, Insertar:572, Insertar:573, Insertar:621, Insertar:624, Insertar:625, Insertar:628, Insertar:629, Insertar:632, Insertar:637, Insertar:638, Insertar:665, Insertar:700, Insertar:701, Insertar:702, Insertar:780, Insertar:781, Insertar:782, Insertar:783, Ángulo:8
307. Lateral Izquierdo Carcasa:1 — Coincidencia:377, Coincidencia:378, Nivelación:54, Coincidencia:387, Coincidencia:388, Coincidencia:389, Coincidencia:392, Insertar:481, Coincidencia:393, Coincidencia:394, Insertar:482, Coincidencia:395, Coincidencia:401, Coincidencia:402, Insertar:533, Insertar:534, Insertar:535, Insertar:536, Insertar:539, Insertar:540, Insertar:545, Insertar:580, Insertar:581, Insertar:582, Insertar:583, Insertar:584, Insertar:585, Insertar:655, Insertar:656, Insertar:657, Insertar:660, Insertar:661, Insertar:664, Insertar:666, Insertar:690, Insertar:691, Insertar:692, Insertar:715, Insertar:716, Insertar:717, Insertar:718, Insertar:719, Insertar:720, Ángulo:4
308. Techo Carcasa:1 — Coincidencia:379, Nivelación:55, Nivelación:56, Coincidencia:382, Coincidencia:396, Insertar:493, Coincidencia:397, Coincidencia:398, Insertar:494, Coincidencia:399, Insertar:537, Insertar:538, Insertar:630, Insertar:631, Insertar:633, Insertar:635, Insertar:653, Insertar:654, Insertar:784, Insertar:785, Insertar:786, Insertar:787, Insertar:788, Insertar:789
309. Culata Carcaza:1 — Coincidencia:380, Coincidencia:381, Coincidencia:382, Insertar:622, Insertar:623, Insertar:626, Insertar:627, Insertar:634, Insertar:636, Insertar:658, Insertar:659, Insertar:662, Insertar:663, Insertar:743, Insertar:744, Insertar:745, Insertar:746
310. Chapon:1 — Insertar:469, Insertar:470, Insertar:733, Insertar:734, Insertar:816, Insertar:817, Insertar:818, Insertar:819, Insertar:830, Insertar:831, Coincidencia:416, Coincidencia:418
311. Separador Lateral:1 — Coincidencia:385, Nivelación:58, Coincidencia:386
312. Separador Lateral:2 — Coincidencia:383, Coincidencia:384, Nivelación:57
313. Cielo raso:1 — Insertar:471, Insertar:472, Coincidencia:404, Insertar:667, Insertar:668, Insertar:669, Insertar:670, Insertar:671, Insertar:672, Insertar:673, Insertar:674, Insertar:675, Insertar:828, Insertar:829, Insertar:854, Insertar:855, Insert:860, Insert:861
314. Puerta Lateral Izquierda:1 — Coincidencia:387, Coincidencia:388, Coincidencia:389
315. Ala 1 Bisagra tipo Libro Grande:1 — Insertar:473, Insertar:474, Insertar:477, Insertar:832, Insertar:833
316. Ala 1 Bisagra tipo Libro Grande:2 — Insertar:475, Insertar:476, Insertar:478, Insertar:834, Insertar:835
317. Ala 2 Bisagra tipo Libro Grande:1 — Insertar:477, Insertar:756, Insertar:772, Insertar:773, Insertar:774
318. Ala 2 Bisagra tipo Libro Grande:2 — Insertar:478, Insertar:755, Insertar:775, Insertar:776, Insertar:777
319. Ala 1 Bisagra tipo T:1 — Coincidencia:392, Insertar:481, Coincidencia:393, Insertar:483, Insertar:722, Insertar:723, Insertar:724
320. Ala 1 Bisagra tipo T:2 — Coincidencia:394, Insertar:482, Coincidencia:395, Insertar:484, Insertar:725, Insertar:726, Insertar:727
321. Ala 2 Bisagra tipo T:1 — Insertar:483, Insertar:812, Insertar:813, Coincidencia:409, Insertar:826
322. Ala 2 Bisagra tipo T:2 — Insertar:484, Insertar:814, Insertar:815, Coincidencia:410, Insertar:827
323. Distanciador para Laterales:1 — Insertar:489
324. Distanciador para Laterales:2 — Insertar:488, Coincidencia:401, Coincidencia:402
325. Distanciador para Laterales:3 — Insertar:487
326. Distanciador para Laterales:4 — Insertar:492
327. Distanciador para Laterales:5 — Insertar:491
328. Distanciador para Laterales:6 — Insertar:490
329. Ala 1 Bisagra tipo Libro Chica:1 — Coincidencia:398, Insertar:494, Coincidencia:399, Insertar:495, Insertar:836, Insertar:837, Insertar:838
330. Ala 1 Bisagra tipo Libro Chica:2 — Coincidencia:396, Insertar:493, Coincidencia:397, Insertar:496, Insertar:839, Insertar:840, Insertar:841
331. Ala 2 Bisagra tipo Libro Chica:1 — Insertar:495, Coincidencia:407, Coincidencia:408, Insertar:767, Insertar:768, Insertar:769
332. Ala 2 Bisagra tipo Libro Chica:2 — Insertar:496, Insertar:757, Insertar:764, Insertar:765, Insertar:766
333. Soporte L:1 — Insertar:521, Insertar:522, Insertar:523, Insertar:524
334. Soporte L:2 — Insertar:513, Insertar:514, Insertar:515, Insertar:516
335. Soporte L:3 — Insertar:505, Insertar:506, Insertar:507, Insertar:508
336. Soporte L:4 — Insertar:497, Insertar:498, Insertar:499, Insertar:500
337. Soporte L:5 — Insertar:501, Insertar:502, Insertar:503, Insertar:504
338. Soporte L:6 — Insertar:509, Insertar:510, Insertar:511, Insertar:512
339. Soporte L:7 — Insertar:517, Insertar:518, Insertar:519, Insertar:520
340. Soporte L:8 — Insertar:525, Insertar:526, Insertar:527, Insertar:528
341. Tuerca remache m4:1 — Insertar:497
342. Tuerca remache m4:2 — Insertar:498, Insertar:540
343. Tuerca remache m4:3 — Insertar:499
344. Tuerca remache m4:4 — Insertar:500, Insertar:539
345. Tuerca remache m4:5 — Insertar:501, Insertar:530
346. Tuerca remache m4:6 — Insertar:502
347. Tuerca remache m4:7 — Insertar:503, Insertar:529
348. Tuerca remache m4:8 — Insertar:504
349. Tuerca remache m4:9 — Insertar:505
350. Tuerca remache m4:10 — Insertar:506, Insertar:542
351. Tuerca remache m4:11 — Insertar:507
352. Tuerca remache m4:12 — Insertar:508, Insertar:541
353. Tuerca remache m4:13 — Insertar:509, Insertar:532
354. Tuerca remache m4:14 — Insertar:510
355. Tuerca remache m4:15 — Insertar:511, Insertar:531
356. Tuerca remache m4:16 — Insertar:512
357. Tuerca remache m4:17 — Insertar:513, Insertar:543
358. Tuerca remache m4:18 — Insertar:514
359. Tuerca remache m4:19 — Insertar:515, Insertar:544
360. Tuerca remache m4:20 — Insertar:516
361. Tuerca remache m4:21 — Insertar:517, Insertar:534
362. Tuerca remache m4:22 — Insertar:518
363. Tuerca remache m4:23 — Insertar:519, Insertar:533
364. Tuerca remache m4:24 — Insertar:520
365. Tuerca remache m4:25 — Insertar:521
366. Tuerca remache m4:26 — Insertar:522, Insertar:538
367. Tuerca remache m4:27 — Insertar:523
368. Tuerca remache m4:28 — Insertar:524, Insertar:537
369. Tuerca remache m4:29 — Insertar:525, Insertar:536
370. Tuerca remache m4:30 — Insertar:526
371. Tuerca remache m4:31 — Insertar:527, Insertar:535
372. Tuerca remache m4:32 — Insertar:528
373. Chapa Base:1 — Insertar:545, Insertar:546, Nivelación:59, Coincidencia:406, Insertar:676
374. Tornillo Allen cabeza botón M6x20mm:41 — Insertar:547
375. Tornillo Allen cabeza botón M6x20mm:42 — Insertar:548
376. Tornillo Allen cabeza botón M6x20mm:43 — Insertar:549
377. Tornillo Allen cabeza botón M6x20mm:53 — Insertar:559
378. Tornillo Allen cabeza botón M6x20mm:54 — Insertar:560
379. Tornillo Allen cabeza botón M6x20mm:55 — Insertar:561
380. Arandela plana tipo A DIN 125 M6:16 — Insertar:583, Insertar:703
381. Arandela plana tipo A DIN 125 M6:17 — Insertar:584, Insertar:704
382. Arandela plana tipo A DIN 125 M6:18 — Insertar:585, Insertar:705
383. Arandela plana tipo A DIN 125 M6:19 — Insertar:559, Insertar:580
384. Arandela plana tipo A DIN 125 M6:20 — Insertar:560, Insertar:581
385. Arandela plana tipo A DIN 125 M6:21 — Insertar:561, Insertar:582
386. Arandela plana tipo A DIN 125 M6:28 — Insertar:571, Insertar:706
387. Arandela plana tipo A DIN 125 M6:29 — Insertar:572, Insertar:707
388. Arandela plana tipo A DIN 125 M6:30 — Insertar:573, Insertar:708
389. Arandela plana tipo A DIN 125 M6:31 — Insertar:547, Insertar:568
390. Arandela plana tipo A DIN 125 M6:32 — Insertar:548, Insertar:569
391. Arandela plana tipo A DIN 125 M6:33 — Insertar:549, Insertar:570
392. Tornillo Allen cabeza botón M4x20mm:7 — Insertar:597
393. Tornillo Allen cabeza botón M4x20mm:8 — Insertar:598
394. Tornillo Allen cabeza botón M4x20mm:9 — Insertar:599
395. Tornillo Allen cabeza botón M4x20mm:10 — Insertar:600
396. Tornillo Allen cabeza botón M4x20mm:11 — Insertar:601
397. Tornillo Allen cabeza botón M4x20mm:12 — Insertar:602
398. Tornillo Allen cabeza botón M4x20mm:13 — Insertar:603
399. Tornillo Allen cabeza botón M4x20mm:14 — Insertar:604
400. Tornillo Allen cabeza botón M4x20mm:15 — Insertar:605
401. Tornillo Allen cabeza botón M4x20mm:16 — Insertar:606
402. Tornillo Allen cabeza botón M4x20mm:17 — Insertar:607
403. Tornillo Allen cabeza botón M4x20mm:18 — Insertar:608
404. Tornillo Allen cabeza botón M4x20mm:19 — Insertar:609
405. Tornillo Allen cabeza botón M4x20mm:20 — Insertar:610
406. Tornillo Allen cabeza botón M4x20mm:21 — Insertar:611
407. Tornillo Allen cabeza botón M4x20mm:22 — Insertar:612
408. Tornillo Allen cabeza botón M4x20mm:23 — Insertar:613, Coincidencia:405
409. Tornillo Allen cabeza botón M4x20mm:24 — Insertar:614
410. Tornillo Allen cabeza botón M4x20mm:27 — Insertar:617
411. Tornillo Allen cabeza botón M4x20mm:28 — Insertar:618
412. Tornillo Allen cabeza botón M4x20mm:29 — Insertar:619
413. Tornillo Allen cabeza botón M4x20mm:30 — Insertar:620
414. Tornillo Allen cabeza botón M4x20mm:31 — Insertar:641
415. Tornillo Allen cabeza botón M4x20mm:32 — Insertar:642
416. Tornillo Allen cabeza botón M4x20mm:33 — Insertar:643
417. Tornillo Allen cabeza botón M4x20mm:34 — Insertar:644
418. Tornillo Allen cabeza botón M4x20mm:35 — Insertar:645
419. Tornillo Allen cabeza botón M4x20mm:36 — Insertar:646
420. Tornillo Allen cabeza botón M4x20mm:37 — Insertar:647
421. Tornillo Allen cabeza botón M4x20mm:38 — Insertar:648
422. Tornillo Allen cabeza botón M4x20mm:39 — Insertar:649
423. Tornillo Allen cabeza botón M4x20mm:40 — Insertar:650
424. Tornillo Allen cabeza botón M4x20mm:41 — Insertar:651
425. Tornillo Allen cabeza botón M4x20mm:42 — Insertar:652
426. Arandela Plana Tipo A DIN 125 - M4:6 — Insertar:641, Insertar:657
427. Arandela Plana Tipo A DIN 125 - M4:7 — Insertar:642, Insertar:658
428. Arandela Plana Tipo A DIN 125 - M4:8 — Insertar:643, Insertar:659
429. Arandela Plana Tipo A DIN 125 - M4:9 — Insertar:644, Insertar:660
430. Arandela Plana Tipo A DIN 125 - M4:10 — Insertar:645, Insertar:661
431. Arandela Plana Tipo A DIN 125 - M4:11 — Insertar:646, Insertar:662
432. Arandela Plana Tipo A DIN 125 - M4:12 — Insertar:647, Insertar:663
433. Arandela Plana Tipo A DIN 125 - M4:13 — Insertar:648, Insertar:664
434. Arandela Plana Tipo A DIN 125 - M4:14 — Insertar:649, Insertar:653
435. Arandela Plana Tipo A DIN 125 - M4:15 — Insertar:650, Insertar:654
436. Arandela Plana Tipo A DIN 125 - M4:16 — Insertar:651, Insertar:655
437. Arandela Plana Tipo A DIN 125 - M4:17 — Insertar:652, Insertar:656
438. Arandela Plana Tipo A DIN 125 - M4:18 — Insertar:597, Insertar:621
439. Arandela Plana Tipo A DIN 125 - M4:19 — Insertar:598, Insertar:622
440. Arandela Plana Tipo A DIN 125 - M4:20 — Insertar:599, Insertar:623
441. Arandela Plana Tipo A DIN 125 - M4:21 — Insertar:600, Insertar:624
442. Arandela Plana Tipo A DIN 125 - M4:22 — Insertar:602, Insertar:626
443. Arandela Plana Tipo A DIN 125 - M4:23 — Insertar:601, Insertar:625
444. Arandela Plana Tipo A DIN 125 - M4:24 — Insertar:603, Insertar:627
445. Arandela Plana Tipo A DIN 125 - M4:25 — Insertar:604, Insertar:628
446. Arandela Plana Tipo A DIN 125 - M4:26 — Insertar:612, Insertar:636
447. Arandela Plana Tipo A DIN 125 - M4:27 — Insertar:611, Insertar:635
448. Arandela Plana Tipo A DIN 125 - M4:28 — Insertar:610, Insertar:634
449. Arandela Plana Tipo A DIN 125 - M4:29 — Insertar:609, Insertar:633
450. Arandela Plana Tipo A DIN 125 - M4:30 — Insertar:608, Insertar:632
451. Arandela Plana Tipo A DIN 125 - M4:31 — Insertar:607, Insertar:631
452. Arandela Plana Tipo A DIN 125 - M4:32 — Insertar:606, Insertar:630
453. Arandela Plana Tipo A DIN 125 - M4:33 — Insertar:605, Insertar:629
454. Arandela Plana Tipo A DIN 125 - M4:34 — Insertar:613, Insertar:665
455. Arandela Plana Tipo A DIN 125 - M4:35 — Insertar:614, Insertar:666
456. Arandela Plana Tipo A DIN 125 - M4:38 — Insertar:617, Insertar:640
457. Arandela Plana Tipo A DIN 125 - M4:39 — Insertar:618, Insertar:639
458. Arandela Plana Tipo A DIN 125 - M4:40 — Insertar:619, Insertar:638
459. Arandela Plana Tipo A DIN 125 - M4:41 — Insertar:620, Insertar:637
460. ISO 4032 M6:1 — Coincidencia:404
461. ISO 4032 M6:2 — Insertar:667
462. ISO 4032 M6:3 — Insertar:668
463. ISO 4032 M6:4 — Insertar:669
464. ISO 4032 M6:5 — Insertar:670
465. ISO 4032 M6:6 — Insertar:672
466. ISO 4032 M6:8 — Insertar:671
467. ISO 4032 M6:9 — Insertar:673
468. ISO 4032 M6:10 — Insertar:674
469. ISO 4032 M6:11 — Insertar:675
470. ISO 4032 M4:1 — Coincidencia:405, Coincidencia:406
471. ISO 4032 M4:2 — Insertar:676
472. Tornillo Allen cabeza botón M6x16mm:20 — Insertar:677
473. Tornillo Allen cabeza botón M6x16mm:21 — Insertar:678
474. Tornillo Allen cabeza botón M6x16mm:22 — Insertar:679
475. Tornillo Allen cabeza botón M6x16mm:23 — Insertar:680
476. Tornillo Allen cabeza botón M6x16mm:24 — Insertar:681
477. Tornillo Allen cabeza botón M6x16mm:25 — Insertar:682
478. Tornillo Allen cabeza botón M6x16mm:26 — Insertar:683
479. Tornillo Allen cabeza botón M6x16mm:27 — Insertar:684
480. Tornillo Allen cabeza botón M6x16mm:28 — Insertar:685
481. Tornillo Allen cabeza botón M6x16mm:29 — Insertar:686
482. Tornillo Allen cabeza botón M6x16mm:30 — Insertar:687
483. Tornillo Allen cabeza botón M6x16mm:31 — Insertar:688
484. Tornillo Allen cabeza botón M6x16mm:32 — Insertar:689
485. Arandela plana tipo A DIN 125 M6:34 — Insertar:677, Insertar:690
486. Arandela plana tipo A DIN 125 M6:35 — Insertar:678, Insertar:691
487. Arandela plana tipo A DIN 125 M6:36 — Insertar:679, Insertar:692
488. Arandela plana tipo A DIN 125 M6:37 — Insertar:680, Insertar:693
489. Arandela plana tipo A DIN 125 M6:38 — Insertar:684, Insertar:700
490. Arandela plana tipo A DIN 125 M6:39 — Insertar:685, Insertar:699
491. Arandela plana tipo A DIN 125 M6:40 — Insertar:686, Insertar:697
492. Arandela plana tipo A DIN 125 M6:41 — Insertar:681, Insertar:694
493. Arandela plana tipo A DIN 125 M6:42 — Insertar:682, Insertar:695
494. Arandela plana tipo A DIN 125 M6:43 — Insertar:683, Insertar:696
495. Arandela plana tipo A DIN 125 M6:44 — Insertar:687, Insertar:702
496. Arandela plana tipo A DIN 125 M6:45 — Insertar:688, Insertar:701
497. Arandela plana tipo A DIN 125 M6:46 — Insertar:689, Insertar:698
498. Tornillo Allen cabeza botón M6x16mm:33 — Insertar:703
499. Tornillo Allen cabeza botón M6x16mm:34 — Insertar:704
500. Tornillo Allen cabeza botón M6x16mm:35 — Insertar:705
501. Tornillo Allen cabeza botón M6x16mm:36 — Insertar:706
502. Tornillo Allen cabeza botón M6x16mm:37 — Insertar:707
503. Tornillo Allen cabeza botón M6x16mm:38 — Insertar:708
504. Arandela plana tipo A DIN 125-M5:1 — Insertar:715, Insertar:721
505. Arandela plana tipo A DIN 125-M5:2 — Insertar:716, Insertar:728
506. Arandela plana tipo A DIN 125-M5:3 — Insertar:717, Insertar:729
507. Arandela plana tipo A DIN 125-M5:4 — Insertar:720, Insertar:732
508. Arandela plana tipo A DIN 125-M5:5 — Insertar:719, Insertar:731
509. Arandela plana tipo A DIN 125-M5:6 — Insertar:718, Insertar:730
510. ISO 4032 M5:1 — Insertar:728
511. ISO 4032 M5:2 — Insertar:729
512. ISO 4032 M5:3 — Insertar:721
513. ISO 4032 M5:4 — Insertar:730
514. ISO 4032 M5:5 — Insertar:731
515. ISO 4032 M5:6 — Insertar:732
516. Tornillo allen cabeza boton M5x16mm:1 — Insertar:723
517. Tornillo allen cabeza boton M5x16mm:2 — Insertar:724
518. Tornillo allen cabeza boton M5x16mm:3 — Insertar:722
519. Tornillo allen cabeza boton M5x16mm:4 — Insertar:725
520. Tornillo allen cabeza boton M5x16mm:5 — Insertar:726
521. Tornillo allen cabeza boton M5x16mm:6 — Insertar:727